# Autodesk Inventor assembly: Coil Designs
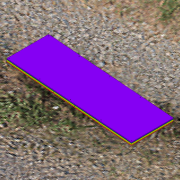
[picture p0: Inventor's stored thumbnail of the model, 180x180]
Saved by Autodesk Inventor 2021 (Build 250183000, 183)
## iProperties
Created: 2022-01-19
Part Number: Coil Designs
Document SubType Name: Assembly
Designer: avan411
Author: avan411
## Documents named in this file (10)
- H:\GitRepos\2021_SRW_RC_CAR\Magnetics\Final Coil Design\CadModels\Coil Designs.iam
- H:\GitRepos\2021_SRW_RC_CAR\Magnetics\Final Coil Design\CadModels\FerriteBar.ipt
- H:\GitRepos\2021_SRW_RC_CAR\Magnetics\Final Coil Design\CadModels\Part2.ipt
- H:\GitRepos\2021_SRW_RC_CAR\Magnetics\Final Coil Design\CadModels\PrimaryCoilFerriteLayer.ipt
- H:\GitRepos\2021_SRW_RC_CAR\Magnetics\Final Coil Design\CadModels\btwnFerriteAndCoil.ipt
- H:\GitRepos\2021_SRW_RC_CAR\Magnetics\Final Coil Design\CadModels\between aluminium and ferrite.ipt
- H:\GitRepos\2021_SRW_RC_CAR\Magnetics\Final Coil Design\CadModels\PrimaryCoilAluminiumLayer.ipt
- H:\GitRepos\2021_SRW_RC_CAR\Magnetics\Final Coil Design\CadModels\aluminium.ipt
- H:\GitRepos\2021_SRW_RC_CAR\Magnetics\Final Coil Design\CadModels\base.ipt
- H:\GitRepos\2021_SRW_RC_CAR\Magnetics\Final Coil Design\CadModels\coil.ipt
## Components (26 placed, 9 different names)
1. PrimaryCoilLayer:1 — Flush:1
2. btwnFerriteAndCoil:1 — Flush:1, Mate:3, Flush:2, Flush:3, Flush:4
3. PrimaryCoifERRITElLayer:2 — Mate:3, Flush:2, Flush:3, Flush:5, Flush:6
4. between aluminium and ferrite:1 — Flush:6, Flush:7, Flush:8, Mate:4, Flush:9, Flush:10
5. PrimaryCoiAluminiumlLayer:3 — Flush:7, Flush:8, Mate:4, Flush:11, Flush:12, Mate:5
6. aluminium:1 — Flush:9, Flush:10
7. base:1 — Flush:11, Flush:12, Mate:5
8. coil:1
9. FerriteBar:2 — Mate:1, Mate:2
10. FerriteBar:1 — Mate:1, Mate:2, Flush:4, Flush:5
11. FerriteBar:3
12. FerriteBar:4
13. FerriteBar:5
14. FerriteBar:6
15. FerriteBar:7
16. FerriteBar:8
17. FerriteBar:9
18. FerriteBar:10
19. FerriteBar:11
20. FerriteBar:12
21. FerriteBar:13
22. FerriteBar:14
23. FerriteBar:15
24. FerriteBar:16
25. FerriteBar:17
26. FerriteBar:18
## Component patterns: (9 elements, first: FerriteBar:2 + FerriteBar:1)
## Relationships (17: Flush 12, Mate 5)
- Mate:1: FerriteBar:2 ↔ FerriteBar:1
- Mate:2: FerriteBar:2 ↔ FerriteBar:1
- Flush:1: PrimaryCoilLayer:1 ↔ btwnFerriteAndCoil:1
- Mate:3: btwnFerriteAndCoil:1 ↔ PrimaryCoifERRITElLayer:2
- Flush:2: btwnFerriteAndCoil:1 ↔ PrimaryCoifERRITElLayer:2
- Flush:3: btwnFerriteAndCoil:1 ↔ PrimaryCoifERRITElLayer:2
- Flush:4 (-60 mm): btwnFerriteAndCoil:1 ↔ FerriteBar:1
- Flush:5: PrimaryCoifERRITElLayer:2 ↔ FerriteBar:1
- Flush:6: PrimaryCoifERRITElLayer:2 ↔ between aluminium and ferrite:1
- Flush:7: between aluminium and ferrite:1 ↔ PrimaryCoiAluminiumlLayer:3
- Flush:8: between aluminium and ferrite:1 ↔ PrimaryCoiAluminiumlLayer:3
- Mate:4: between aluminium and ferrite:1 ↔ PrimaryCoiAluminiumlLayer:3
- Flush:9: between aluminium and ferrite:1 ↔ aluminium:1
- Flush:10: between aluminium and ferrite:1 ↔ aluminium:1
- Flush:11: PrimaryCoiAluminiumlLayer:3 ↔ base:1
- Flush:12: PrimaryCoiAluminiumlLayer:3 ↔ base:1
- Mate:5: PrimaryCoiAluminiumlLayer:3 ↔ base:1
